# Autodesk Inventor assembly: Assembly1
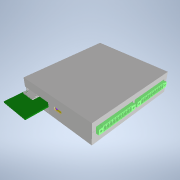
[picture p0: Inventor's stored thumbnail of the model, 180x180]
Saved by Autodesk Inventor 2022 (Build 260153070, 153G)
## iProperties
Created: 2021-07-15
Part Number: Assembly1
Document SubType Name: Assembly
Designer: Eakawit_kor
Author: Eakawit_kor
## Documents named in this file (5)
- C:\Users\Eakawit_kor\OneDrive - EASTWATER GROUP\Workspace\4_UUControl\UUControl\1_Hardware\02_Assembly\Assembly1.iam
- C:\Users\Eakawit_kor\OneDrive - EASTWATER GROUP\Workspace\4_UUControl\UUControl\2_Electonic\OUTJOB\DesignData\ExportSTEP\ExportSTEP UU001-A0_UU Control Board.iam
- C:\Users\Eakawit_kor\OneDrive - EASTWATER GROUP\Workspace\4_UUControl\UUControl\1_Hardware\01_Part\BaseCase.ipt
- C:\Users\Eakawit_kor\OneDrive - EASTWATER GROUP\Workspace\4_UUControl\UUCommunication\2_Electonic\UC001_LTE\OUTJOB\DesignData\ExportSTEP\ExportSTEP UC001-A0_UUC-LTE.iam
- C:\Users\Eakawit_kor\OneDrive - EASTWATER GROUP\Workspace\4_UUControl\UUControl\1_Hardware\01_Part\TopCase.ipt
## Components (4 placed, 4 different names)
1. ExportSTEP UU001-A0_UU Control Board:1 [sub-assembly] — Mate:1, Mate:3, Mate:9
2. BaseCase:1 — Mate:1, Mate:3, Mate:4, Mate:5, Mate:6, Mate:7, Mate:8, Mate:9, Mate:10, Flush:1, Flush:2
3. ExportSTEP UC001-A0_UUC-LTE:1 [sub-assembly] — Mate:6, Mate:7, Mate:8
4. TopCase:1 — Flush:1, Flush:2
## Relationships (11: Mate 9, Flush 2)
- Mate:1: ExportSTEP UU001-A0_UU Control Board:1 ↔ BaseCase:1
- Mate:3: ExportSTEP UU001-A0_UU Control Board:1 ↔ BaseCase:1
- Mate:4: BaseCase:1
- Mate:5: BaseCase:1
- Mate:6: BaseCase:1 ↔ ExportSTEP UC001-A0_UUC-LTE:1
- Mate:7: BaseCase:1 ↔ ExportSTEP UC001-A0_UUC-LTE:1
- Mate:8: BaseCase:1 ↔ ExportSTEP UC001-A0_UUC-LTE:1
- Mate:9: ExportSTEP UU001-A0_UU Control Board:1 ↔ BaseCase:1
- Mate:10: BaseCase:1
- Flush:1: BaseCase:1 ↔ TopCase:1
- Flush:2: BaseCase:1 ↔ TopCase:1
